# Autodesk Inventor assembly: BotV1
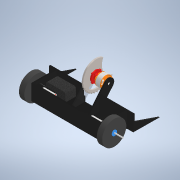
[picture p0: Inventor's stored thumbnail of the model, 180x180]
Saved by Autodesk Inventor 2020 (Build 240168000, 168)
## iProperties
Created: 2023-11-26
Part Number: BotV1
Document SubType Name: Assembly
Designer: smz3rm
Mass: 366.58 g
Surface Area: 1094.11 cm^2
Volume: 225.239 cm^3
Density: 1.62752 g/cm^3
Author: smz3rm
## Documents named in this file (11)
- C:\Users\smz3rm\OneDrive - BP\Documents\DigitalTwin\Models\BattleBot\BotV1.iam
- C:\Users\smz3rm\OneDrive - BP\Documents\DigitalTwin\Models\BattleBot\BodyV2.ipt
- C:\Users\smz3rm\OneDrive - BP\Documents\DigitalTwin\Models\BattleBot\BatteryV1.ipt
- C:\Users\smz3rm\OneDrive - BP\Documents\DigitalTwin\Models\BattleBot\WheelV1.ipt
- C:\Users\smz3rm\OneDrive - BP\Documents\DigitalTwin\Models\BattleBot\DriveMotorV2.ipt
- C:\Users\smz3rm\OneDrive - BP\Documents\DigitalTwin\Models\BattleBot\HubV2.ipt
- C:\Users\smz3rm\OneDrive - BP\Documents\DigitalTwin\Models\BattleBot\BladeHubV1.ipt
- C:\Users\smz3rm\OneDrive - BP\Documents\DigitalTwin\Models\BattleBot\WeaponV2.ipt
- C:\Users\smz3rm\OneDrive - BP\Documents\DigitalTwin\Models\BattleBot\WeaponMotorV1.ipt
- C:\Users\smz3rm\OneDrive - BP\Documents\DigitalTwin\Models\BattleBot\WeaponBearingV1.ipt
- C:\Users\smz3rm\OneDrive - BP\Documents\DigitalTwin\Models\BattleBot\WeaponStandoffBearingV1.ipt
## Components (14 placed, 10 different names)
1. BodyV2:1 — Mate:11, Mate:12, Mate:13, Mate:14, Mate:15, Mate:16, Mate:17, Mate:18, Mate:19, Mate:26, Mate:27, Mate:36, Mate:39, Mate:40
2. BatteryV1:1 — Mate:11, Mate:12, Mate:13
3. DriveMotorV2:1 — Mate:14, Mate:15, Mate:16, Mate:25
4. DriveMotorV2:2 — Mate:17, Mate:18, Mate:19, Mate:24
5. HubV2:1 — Mate:20, Mate:21, Mate:24, Mate:27
6. WheelV1:1 — Mate:20, Mate:21
7. HubV2:2 — Mate:22, Mate:23, Mate:25, Mate:26
8. WheelV1:2 — Mate:22, Mate:23
9. BladeHubV1:1 — Mate:28, Mate:29, Mate:30, Mate:31, Mate:32, Mate:33, Mate:35
10. WeaponV2:1 — Mate:28, Mate:29, Mate:30, Mate:31
11. WeaponMotorV1:1 — Mate:32, Mate:33, Mate:34, Mate:41, Mate:42
12. WeaponBearingV1:1 — Mate:34, Mate:35, Mate:37, Mate:38
13. WeaponStandoffBearingV1:1 — Mate:36, Mate:37, Mate:38, Mate:39, Mate:40
14. WeaponStandoffBearingV1:2 — Mate:41, Mate:42
## Relationships (32: Mate 32)
- Mate:11: BodyV2:1 ↔ BatteryV1:1
- Mate:12: BodyV2:1 ↔ BatteryV1:1
- Mate:13: BodyV2:1 ↔ BatteryV1:1
- Mate:14: BodyV2:1 ↔ DriveMotorV2:1
- Mate:15: BodyV2:1 ↔ DriveMotorV2:1
- Mate:16: BodyV2:1 ↔ DriveMotorV2:1
- Mate:17: BodyV2:1 ↔ DriveMotorV2:2
- Mate:18: BodyV2:1 ↔ DriveMotorV2:2
- Mate:19: BodyV2:1 ↔ DriveMotorV2:2
- Mate:20: HubV2:1 ↔ WheelV1:1
- Mate:21: HubV2:1 ↔ WheelV1:1
- Mate:22: HubV2:2 ↔ WheelV1:2
- Mate:23: HubV2:2 ↔ WheelV1:2
- Mate:24: DriveMotorV2:2 ↔ HubV2:1
- Mate:25: DriveMotorV2:1 ↔ HubV2:2
- Mate:26: BodyV2:1 ↔ HubV2:2
- Mate:27: BodyV2:1 ↔ HubV2:1
- Mate:28: BladeHubV1:1 ↔ WeaponV2:1
- Mate:29: BladeHubV1:1 ↔ WeaponV2:1
- Mate:30: BladeHubV1:1 ↔ WeaponV2:1
- Mate:31: BladeHubV1:1 ↔ WeaponV2:1
- Mate:32: BladeHubV1:1 ↔ WeaponMotorV1:1
- Mate:33: BladeHubV1:1 ↔ WeaponMotorV1:1
- Mate:34: WeaponMotorV1:1 ↔ WeaponBearingV1:1
- Mate:35: BladeHubV1:1 ↔ WeaponBearingV1:1
- Mate:36: BodyV2:1 ↔ WeaponStandoffBearingV1:1
- Mate:37: WeaponBearingV1:1 ↔ WeaponStandoffBearingV1:1
- Mate:38: WeaponBearingV1:1 ↔ WeaponStandoffBearingV1:1
- Mate:39: BodyV2:1 ↔ WeaponStandoffBearingV1:1
- Mate:40: BodyV2:1 ↔ WeaponStandoffBearingV1:1
- Mate:41: WeaponMotorV1:1 ↔ WeaponStandoffBearingV1:2
- Mate:42: WeaponMotorV1:1 ↔ WeaponStandoffBearingV1:2
